# Autodesk Inventor assembly: YAxis_Carriage
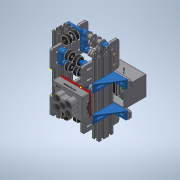
[picture p0: Inventor's stored thumbnail of the model, 180x180]
Saved by Autodesk Inventor 2021 (Build 250183000, 183)
## iProperties
Created: 2021-02-02
Part Number: YAxis_Carriage
Document SubType Name: Assembly
Designer: Jorian Brusind
Author: Jorian Brusind
## Documents named in this file (18)
- C:\Users\Jorian Brusind\Documents\GitHub\PersonalProjects\HyperRail\Inventor Files\YAxis_Carriage.iam
- C:\Users\Jorian Brusind\Documents\GitHub\PersonalProjects\HyperRail\Inventor Files\SmallBelt_Pulley.ipt
- C:\Users\Jorian Brusind\Documents\GitHub\PersonalProjects\Inventor Projects\Useful models\Metric bolt\Bolt M3 30mm.ipt
- C:\Users\Jorian Brusind\Documents\GitHub\PersonalProjects\HyperRail\Inventor Files\small_belt_loop.ipt
- C:\Users\Jorian Brusind\Documents\GitHub\PersonalProjects\HyperRail\PCB Files\Integrated Stepper Motor Driver\ExportSTEP\Main.iam
- C:\Users\Jorian Brusind\Documents\GitHub\PersonalProjects\HyperRail\Inventor Files\rededge-micasense-1.snapshot.3\PND_CAM_MSRE.ipt
- C:\Users\Jorian Brusind\Documents\GitHub\PersonalProjects\HyperRail\Inventor Files\NEMA17_Shroud.ipt
- C:\Users\Jorian Brusind\Documents\GitHub\PersonalProjects\HyperRail\Inventor Files\Buffer.iam
- C:\Users\Jorian Brusind\Documents\GitHub\PersonalProjects\HyperRail\Inventor Files\X_Carriage_V2_0.iam
- C:\Users\Jorian Brusind\Documents\GitHub\PersonalProjects\HyperRail\Inventor Files\X_CarriageR_V2_0.iam
- C:\Users\Jorian Brusind\Documents\GitHub\PersonalProjects\HyperRail\Inventor Files\X_CarriageR_V2_1.iam
- C:\Users\Jorian Brusind\Documents\GitHub\PersonalProjects\HyperRail\Inventor Files\X_Carriage_V2_1.iam
- C:\Users\Jorian Brusind\Documents\GitHub\PersonalProjects\Inventor Projects\Useful models\8020_Sets\IPT_20_Series\IPT_20_Series\20-2040_200mm.ipt
- C:\Users\Jorian Brusind\Documents\GitHub\PersonalProjects\HyperRail\Inventor Files\10mm_Idle_Pulley_3M.ipt
- C:\Users\Jorian Brusind\Documents\GitHub\PersonalProjects\HyperRail\Inventor Files\McMaster Files\Hex Standoffs\95947A725_Aluminum Female Threaded Hex Standoff.ipt
- C:\Users\Jorian Brusind\Documents\GitHub\PersonalProjects\Inventor Projects\Useful models\Metric bolt\Bolt M5 45mm.ipt
- C:\Users\Jorian Brusind\Documents\GitHub\PersonalProjects\HyperRail\Inventor Files\nema17-x-40-1.snapshot.7\NEMA17 x 40.ipt
- C:\Users\Jorian Brusind\Documents\GitHub\PersonalProjects\HyperRail\Inventor Files\RightAngle_Bracket.ipt
## Components (33 placed, 17 different names)
1. SmallBelt_Pulley:1 — Mate:37, Flush:94, Mate:208, Flush:102, Flush:103
2. small_belt_loop:1 — Mate:37, Mate:213, Angle:1
3. Main:1 [sub-assembly] — Mate:209, Mate:210, Mate:211
4. PND_CAM_MSRE:1 — Mate:188, Flush:95, Mate:189
5. 20-2040_200mm:1 — Flush:74, Flush:75, Mate:151, Mate:157, Mate:158, Flush:76, Flush:77, Flush:78, Flush:79, Mate:161, Flush:80, Mate:175, Flush:89, Mate:188
6. 20-2040_200mm:2 — Flush:74, Flush:75, Mate:155, Mate:156, Mate:160, Mate:174, Flush:95, Mate:223, Mate:224, Mate:227
7. X_CarriageR_V2_0:4 [sub-assembly] — Mate:161, Flush:80, Mate:162, Mate:163, Flush:85, Mate:166, Mate:167, Flush:86, Flush:90, Mate:186, Mate:191, Mate:192, Mate:200, Mate:201, Mate:202
8. X_Carriage_V2_1:3 [sub-assembly] — Mate:160, Mate:163, Flush:85, Mate:166, Mate:167, Mate:186, Mate:190, Mate:193, Mate:198, Mate:199, Mate:205, Flush:103
9. Buffer:4 [sub-assembly] — Mate:157, Flush:76, Flush:77, Mate:162
10. Buffer:5 [sub-assembly] — Mate:158, Flush:78, Flush:79
11. Bolt M3 30mm:2 — Mate:183, Mate:184, Mate:219
12. X_Carriage_V2_0:1 [sub-assembly] — Mate:175, Flush:86, Flush:87, Flush:88, Flush:89, Mate:176, Flush:90, Mate:177, Mate:187, Mate:194, Mate:196, Mate:206, Mate:207
13. X_CarriageR_V2_1:1 [sub-assembly] — Mate:174, Flush:87, Flush:88, Mate:176, Mate:177, Mate:187, Mate:189, Mate:195, Mate:197, Mate:203, Mate:204, Mate:217
14. 10mm_Idle_Pulley_3M:1 — Flush:93, Mate:222
15. 10mm_Idle_Pulley_3M:2 — Flush:91, Mate:220
16. 10mm_Idle_Pulley_3M:3 — Flush:92, Mate:221
17. 10mm_Idle_Pulley_3M:4 — Flush:91, Flush:92, Flush:93, Flush:94, Mate:183, Mate:184
18. 95947A725_Aluminum Female Threaded Hex Standoff:1 — Mate:190, Mate:191
19. 95947A725_Aluminum Female Threaded Hex Standoff:2 — Mate:192, Mate:193
20. 95947A725_Aluminum Female Threaded Hex Standoff:3 — Mate:194, Mate:195
21. 95947A725_Aluminum Female Threaded Hex Standoff:4 — Mate:196, Mate:197
22. Bolt M5 45mm:1 — Mate:201, Flush:96, Mate:202, Flush:101
23. Bolt M5 45mm:2 — Mate:198, Flush:97
24. Bolt M5 45mm:3 — Mate:207, Flush:100, Flush:101
25. Bolt M5 45mm:4 — Mate:206, Flush:100
26. Bolt M5 45mm:5 — Mate:200, Flush:96
27. Bolt M5 45mm:6 — Mate:203, Flush:98, Flush:99
28. Bolt M5 45mm:7 — Mate:204, Flush:98
29. Bolt M5 45mm:8 — Mate:199, Flush:97, Flush:99, Mate:205
30. NEMA17 x 40:1 — Mate:208, Mate:209, Mate:210, Mate:211, Mate:213, Flush:102, Mate:214, Mate:215, Mate:216
31. NEMA17_Shroud:1 — Mate:214, Mate:215, Mate:216, Mate:217, Mate:219, Mate:220, Mate:221, Mate:222, Angle:1, Mate:225, Mate:226, Flush:104, Flush:105, Mate:227
32. RightAngle_Bracket:1 — Mate:224, Mate:226, Flush:104
33. RightAngle_Bracket:2 — Mate:223, Mate:225, Flush:105
## Relationships (87: Mate 58, Flush 28, Angle 1)
- Mate:37 (2 mm): SmallBelt_Pulley:1 ↔ small_belt_loop:1
- Flush:74: 20-2040_200mm:1 ↔ 20-2040_200mm:2
- Flush:75: 20-2040_200mm:1 ↔ 20-2040_200mm:2
- Mate:151: 20-2040_200mm:1
- Mate:155: 20-2040_200mm:2
- Mate:156: 20-2040_200mm:2
- Mate:157: 20-2040_200mm:1 ↔ Buffer:4
- Mate:158: 20-2040_200mm:1 ↔ Buffer:5
- Flush:76: 20-2040_200mm:1 ↔ Buffer:4
- Flush:77: 20-2040_200mm:1 ↔ Buffer:4
- Flush:78: 20-2040_200mm:1 ↔ Buffer:5
- Flush:79: 20-2040_200mm:1 ↔ Buffer:5
- Mate:160: 20-2040_200mm:2 ↔ X_Carriage_V2_1:3
- Mate:161: 20-2040_200mm:1 ↔ X_CarriageR_V2_0:4
- Flush:80: 20-2040_200mm:1 ↔ X_CarriageR_V2_0:4
- Mate:162 (4 mm): X_CarriageR_V2_0:4 ↔ Buffer:4
- Mate:163: X_CarriageR_V2_0:4 ↔ X_Carriage_V2_1:3
- Flush:85: X_CarriageR_V2_0:4 ↔ X_Carriage_V2_1:3
- Mate:166 (10 mm): X_CarriageR_V2_0:4 ↔ X_Carriage_V2_1:3
- Mate:167: X_CarriageR_V2_0:4 ↔ X_Carriage_V2_1:3
- Mate:174: 20-2040_200mm:2 ↔ X_CarriageR_V2_1:1
- Mate:175: 20-2040_200mm:1 ↔ X_Carriage_V2_0:1
- Flush:86: X_CarriageR_V2_0:4 ↔ X_Carriage_V2_0:1
- Flush:87: X_Carriage_V2_0:1 ↔ X_CarriageR_V2_1:1
- Flush:88: X_Carriage_V2_0:1 ↔ X_CarriageR_V2_1:1
- Flush:89: 20-2040_200mm:1 ↔ X_Carriage_V2_0:1
- Mate:176: X_Carriage_V2_0:1 ↔ X_CarriageR_V2_1:1
- Flush:90: X_CarriageR_V2_0:4 ↔ X_Carriage_V2_0:1
- Mate:177: X_Carriage_V2_0:1 ↔ X_CarriageR_V2_1:1
- Flush:91: 10mm_Idle_Pulley_3M:2 ↔ 10mm_Idle_Pulley_3M:4
- Flush:92: 10mm_Idle_Pulley_3M:3 ↔ 10mm_Idle_Pulley_3M:4
- Flush:93: 10mm_Idle_Pulley_3M:1 ↔ 10mm_Idle_Pulley_3M:4
- Flush:94: SmallBelt_Pulley:1 ↔ 10mm_Idle_Pulley_3M:4
- Mate:183: Bolt M3 30mm:2 ↔ 10mm_Idle_Pulley_3M:4
- Mate:184: Bolt M3 30mm:2 ↔ 10mm_Idle_Pulley_3M:4
- Mate:186: X_CarriageR_V2_0:4 ↔ X_Carriage_V2_1:3
- Mate:187: X_Carriage_V2_0:1 ↔ X_CarriageR_V2_1:1
- Mate:188 (20 mm): PND_CAM_MSRE:1 ↔ 20-2040_200mm:1
- Flush:95: PND_CAM_MSRE:1 ↔ 20-2040_200mm:2
- Mate:189 (0.5 mm): PND_CAM_MSRE:1 ↔ X_CarriageR_V2_1:1
- Mate:190: X_Carriage_V2_1:3 ↔ 95947A725_Aluminum Female Threaded Hex Standoff:1
- Mate:191: X_CarriageR_V2_0:4 ↔ 95947A725_Aluminum Female Threaded Hex Standoff:1
- Mate:192: X_CarriageR_V2_0:4 ↔ 95947A725_Aluminum Female Threaded Hex Standoff:2
- Mate:193: X_Carriage_V2_1:3 ↔ 95947A725_Aluminum Female Threaded Hex Standoff:2
- Mate:194: X_Carriage_V2_0:1 ↔ 95947A725_Aluminum Female Threaded Hex Standoff:3
- Mate:195: X_CarriageR_V2_1:1 ↔ 95947A725_Aluminum Female Threaded Hex Standoff:3
- Mate:196: X_Carriage_V2_0:1 ↔ 95947A725_Aluminum Female Threaded Hex Standoff:4
- Mate:197: X_CarriageR_V2_1:1 ↔ 95947A725_Aluminum Female Threaded Hex Standoff:4
- Mate:198: X_Carriage_V2_1:3 ↔ Bolt M5 45mm:2
- Mate:199: X_Carriage_V2_1:3 ↔ Bolt M5 45mm:8
- Mate:200: X_CarriageR_V2_0:4 ↔ Bolt M5 45mm:5
- Mate:201: X_CarriageR_V2_0:4 ↔ Bolt M5 45mm:1
- Flush:96: Bolt M5 45mm:1 ↔ Bolt M5 45mm:5
- Mate:202: X_CarriageR_V2_0:4 ↔ Bolt M5 45mm:1
- Flush:97: Bolt M5 45mm:2 ↔ Bolt M5 45mm:8
- Mate:203: X_CarriageR_V2_1:1 ↔ Bolt M5 45mm:6
- Mate:204: X_CarriageR_V2_1:1 ↔ Bolt M5 45mm:7
- Flush:98: Bolt M5 45mm:6 ↔ Bolt M5 45mm:7
- Flush:99: Bolt M5 45mm:6 ↔ Bolt M5 45mm:8
- Mate:205: X_Carriage_V2_1:3 ↔ Bolt M5 45mm:8
- Mate:206: X_Carriage_V2_0:1 ↔ Bolt M5 45mm:4
- Mate:207: X_Carriage_V2_0:1 ↔ Bolt M5 45mm:3
- Flush:100: Bolt M5 45mm:3 ↔ Bolt M5 45mm:4
- Flush:101: Bolt M5 45mm:1 ↔ Bolt M5 45mm:3
- Mate:208: SmallBelt_Pulley:1 ↔ NEMA17 x 40:1
- Mate:209: Main:1 ↔ NEMA17 x 40:1
- Mate:210: Main:1 ↔ NEMA17 x 40:1
- Mate:211 (8 mm): Main:1 ↔ NEMA17 x 40:1
- Mate:213: small_belt_loop:1 ↔ NEMA17 x 40:1
- Flush:102: SmallBelt_Pulley:1 ↔ NEMA17 x 40:1
- Flush:103: SmallBelt_Pulley:1 ↔ X_Carriage_V2_1:3
- Mate:214: NEMA17 x 40:1 ↔ NEMA17_Shroud:1
- Mate:215: NEMA17 x 40:1 ↔ NEMA17_Shroud:1
- Mate:216: NEMA17 x 40:1 ↔ NEMA17_Shroud:1
- Mate:217 (3 mm): X_CarriageR_V2_1:1 ↔ NEMA17_Shroud:1
- Mate:219: Bolt M3 30mm:2 ↔ NEMA17_Shroud:1
- Mate:220: 10mm_Idle_Pulley_3M:2 ↔ NEMA17_Shroud:1
- Mate:221: 10mm_Idle_Pulley_3M:3 ↔ NEMA17_Shroud:1
- Mate:222: 10mm_Idle_Pulley_3M:1 ↔ NEMA17_Shroud:1
- Angle:1 (0 deg): small_belt_loop:1 ↔ NEMA17_Shroud:1
- Mate:223: 20-2040_200mm:2 ↔ RightAngle_Bracket:2
- Mate:224: 20-2040_200mm:2 ↔ RightAngle_Bracket:1
- Mate:225: NEMA17_Shroud:1 ↔ RightAngle_Bracket:2
- Mate:226: NEMA17_Shroud:1 ↔ RightAngle_Bracket:1
- Flush:104: NEMA17_Shroud:1 ↔ RightAngle_Bracket:1
- Flush:105: NEMA17_Shroud:1 ↔ RightAngle_Bracket:2
- Mate:227: 20-2040_200mm:2 ↔ NEMA17_Shroud:1
